# Autodesk Inventor assembly: print of A parts
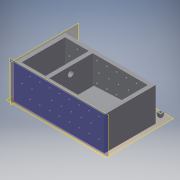
[picture p0: Inventor's stored thumbnail of the model, 180x180]
Saved by Autodesk Inventor 2019 (Build 230136000, 136)
## iProperties
Created: 2018-07-24
Part Number: print of A parts
Document SubType Name: Assembly
Designer: email
Author: email
## Documents named in this file (3)
- D:\College\smarterCampus\smarterCampus\print of A parts.iam
- D:\College\smarterCampus\smarterCampus\bottomA.ipt
- D:\College\smarterCampus\smarterCampus\Press  Fit Foot A.ipt
## Components (5 placed, 2 different names)
1. bottomA:1 — Mate:1, Mate:2, Mate:3
2. Press  Fit Foot A:1 — Mate:4, Flush:1
3. Press  Fit Foot A:2 — Flush:1, Flush:2, Flush:3
4. Press  Fit Foot A:3 — Flush:2
5. Press  Fit Foot A:4 — Flush:3
## Relationships (7: Mate 4, Flush 3)
- Mate:1: bottomA:1
- Mate:2: bottomA:1
- Mate:3: bottomA:1
- Mate:4: Press  Fit Foot A:1
- Flush:1: Press  Fit Foot A:1 ↔ Press  Fit Foot A:2
- Flush:2: Press  Fit Foot A:2 ↔ Press  Fit Foot A:3
- Flush:3: Press  Fit Foot A:2 ↔ Press  Fit Foot A:4
